# Autodesk Inventor assembly: Firing Pin
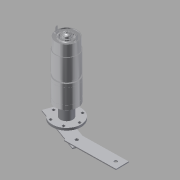
[picture p0: Inventor's stored thumbnail of the model, 180x180]
Saved by Autodesk Inventor 2013 (Build 170138000, 138)
## iProperties
Created: 2013-01-27
Part Number: Firing Pin
Document SubType Name: Assembly
Designer: carneeki
Author: carneeki
## Documents named in this file (6)
- C:\Autodesk\gruntmaster6000-cad\Shooter\Firing Pin\Firing Pin.iam
- C:\Autodesk\gruntmaster6000-cad\Shooter\Firing Pin\Part4.ipt
- C:\Autodesk\gruntmaster6000-cad\Shooter\Firing Pin\10mm-key-hub-am-0985.ipt
- C:\Autodesk\gruntmaster6000-cad\Shooter\Firing Pin\Theta Bar.ipt
- C:\Autodesk\gruntmaster6000-cad\Imported Components\Motors\PG27\PG27.ipt
- C:\Autodesk\gruntmaster6000-cad\Imported Components\Motors\4x4x12 PG-27 Machine Key.ipt
## Components (6 placed, 6 different names)
1. Ram — Insert:2, Mate:9
2. PG27:1 — Mate:7, Flush:1, Insert:5, Mate:8
3. 4x4x12 PG-27 Machine Key:1 — Mate:7, Flush:1, Mate:8
4. 10mm-key-hub-am-0985:1 — Insert:4, Insert:6
5. Z Bar — Insert:2, Insert:4
6. Mount Bar — Insert:5, Insert:6, Mate:9
## Relationships (8: Insert 4, Mate 3, Flush 1)
- Insert:2: Ram ↔ Z Bar
- Mate:7: PG27:1 ↔ 4x4x12 PG-27 Machine Key:1
- Insert:4: 10mm-key-hub-am-0985:1 ↔ Z Bar
- Flush:1: PG27:1 ↔ 4x4x12 PG-27 Machine Key:1
- Insert:5: PG27:1 ↔ Mount Bar
- Mate:8: PG27:1 ↔ 4x4x12 PG-27 Machine Key:1
- Insert:6: 10mm-key-hub-am-0985:1 ↔ Mount Bar
- Mate:9: Ram ↔ Mount Bar
